# Autodesk Inventor assembly: chain test
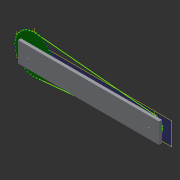
[picture p0: Inventor's stored thumbnail of the model, 180x180]
Saved by Autodesk Inventor 2019 (Build 230136000, 136)
## iProperties
Created: 2020-06-02
Part Number: chain test
Document SubType Name: Assembly
Designer: 18186
Author: 18186
## Documents named in this file (4)
- C:\Users\18186\Desktop\Important Shit\Michael Goldberg Portfolio\CAD Portfolio\IPT Files\Bike\chain test.iam
- C:\Users\18186\Desktop\Important Shit\Michael Goldberg Portfolio\CAD Portfolio\IPT Files\Bike\Sprocket Chain Positioning 1.ipt
- C:\Users\18186\Desktop\Important Shit\Michael Goldberg Portfolio\CAD Portfolio\IPT Files\Bike\Sprocket Chain Positioning 2.ipt
- C:\Users\18186\Desktop\Important Shit\Michael Goldberg Portfolio\CAD Portfolio\IPT Files\Bike\test rack.ipt
## Components (3 placed, 3 different names)
1. Sprocket Chain Positioning 1:1 — Flush:1, Mate:1
2. Sprocket Chain Positioning 2:1 — Flush:1, Mate:2, Flush:2
3. test rack:1 — Mate:1, Mate:2, Flush:2, Flush:3
## Relationships (5: Flush 3, Mate 2)
- Flush:1: Sprocket Chain Positioning 1:1 ↔ Sprocket Chain Positioning 2:1
- Mate:1: Sprocket Chain Positioning 1:1 ↔ test rack:1
- Mate:2: Sprocket Chain Positioning 2:1 ↔ test rack:1
- Flush:2: Sprocket Chain Positioning 2:1 ↔ test rack:1
- Flush:3 (12.7 mm): test rack:1
